# Autodesk Inventor assembly: chassis weldment top
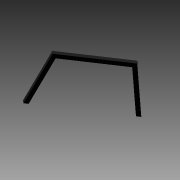
[picture p0: Inventor's stored thumbnail of the model, 180x180]
Saved by Autodesk Inventor 2012 (Build 160160000, 160)
## iProperties
Created: 2011-09-30
Part Number: chassis weldment top
Document SubType Name: Weldment
Designer: Antonella
Weld Material: Welded Aluminum-6061
Author: Antonella
## Documents named in this file (3)
- C:\Users\Antonella\Documents\GCC Robotics 2012 - Mechanical\Robot 2.0\Chassis\chassis weldment top.iam
- C:\Users\Antonella\Documents\GCC Robotics 2012 - Mechanical\Robot 2.0\Chassis\top frame member crossbrace.ipt
- C:\Users\Antonella\Documents\GCC Robotics 2012 - Mechanical\Robot 2.0\Chassis\top frame member back support.ipt
## Components (3 placed, 2 different names)
1. top frame member crossbrace:2 — Mate:8, Flush:6, Mate:9, Mate:10, Flush:7, Mate:11
2. top frame member back support:1 — Mate:8, Flush:6, Mate:9
3. top frame member back support:2 — Mate:10, Flush:7, Mate:11
## Relationships (6: Mate 4, Flush 2)
- Mate:8: top frame member crossbrace:2 ↔ top frame member back support:1
- Flush:6: top frame member crossbrace:2 ↔ top frame member back support:1
- Mate:9: top frame member crossbrace:2 ↔ top frame member back support:1
- Mate:10: top frame member crossbrace:2 ↔ top frame member back support:2
- Flush:7: top frame member crossbrace:2 ↔ top frame member back support:2
- Mate:11: top frame member crossbrace:2 ↔ top frame member back support:2
